# Autodesk Inventor assembly: Structure
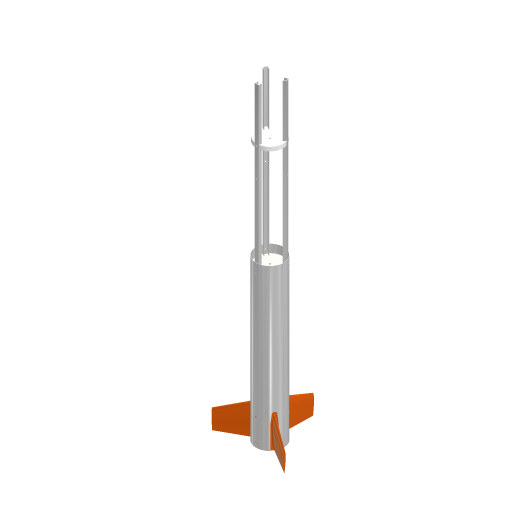
[picture p0: Inventor's stored thumbnail of the model, 512x512]
Saved by Autodesk Inventor 2024 (Build 280153000, 153)
## iProperties
Created: 2023-12-30
Part Number: Structure
Document SubType Name: Assembly
Designer: Jamie
Author: Jamie
## Documents named in this file (6)
- C:\Users\Jamie\Documents\Uni\DARE\Scrambler-2-CAD\Autodesk\Structure.iam
- C:\Users\Jamie\Documents\Uni\DARE\Scrambler-2-CAD\Autodesk\Engine bulkhead.ipt
- C:\Users\Jamie\Documents\Uni\DARE\Scrambler-2-CAD\Autodesk\Engine skin sheet metal.ipt
- C:\Users\Jamie\Documents\Uni\DARE\Scrambler-2-CAD\Autodesk\Stringer.ipt
- C:\Users\Jamie\Documents\Uni\DARE\Scrambler-2-CAD\Autodesk\Parachute bulkhead.ipt
- C:\Users\Jamie\Documents\Uni\DARE\Scrambler-2-CAD\Autodesk\Fins.ipt
## Components (7 placed, 5 different names)
1. Engine bulkhead:1 — Mate:1, Mate:2, Mate:6, Mate:7, Mate:8
2. Engine skin sheet metal:1 — Mate:1, Mate:2, Mate:3, Mate:4, Mate:5, Mate:14, Mate:16, Mate:17
3. Stringer:1 — Mate:4, Mate:7, Mate:12
4. Stringer:2 — Mate:3, Mate:6, Mate:13, Mate:15
5. Stringer:3 — Mate:5, Mate:8, Mate:11
6. Parachute bulkhead:1 — Mate:11, Mate:12, Mate:13, Mate:14, Mate:15
7. Fins:1 — Mate:16, Mate:17
## Relationships (15: Mate 15)
- Mate:1: Engine bulkhead:1 ↔ Engine skin sheet metal:1
- Mate:2: Engine bulkhead:1 ↔ Engine skin sheet metal:1
- Mate:3: Engine skin sheet metal:1 ↔ Stringer:2
- Mate:4: Engine skin sheet metal:1 ↔ Stringer:1
- Mate:5: Engine skin sheet metal:1 ↔ Stringer:3
- Mate:6: Engine bulkhead:1 ↔ Stringer:2
- Mate:7: Engine bulkhead:1 ↔ Stringer:1
- Mate:8: Engine bulkhead:1 ↔ Stringer:3
- Mate:11 (0.5 mm): Stringer:3 ↔ Parachute bulkhead:1
- Mate:12 (0.5 mm): Stringer:1 ↔ Parachute bulkhead:1
- Mate:13 (0.5 mm): Stringer:2 ↔ Parachute bulkhead:1
- Mate:14: Engine skin sheet metal:1 ↔ Parachute bulkhead:1
- Mate:15: Stringer:2 ↔ Parachute bulkhead:1
- Mate:16: Engine skin sheet metal:1 ↔ Fins:1
- Mate:17: Engine skin sheet metal:1 ↔ Fins:1
